# Autodesk Inventor assembly: OUTK_000_Assembly
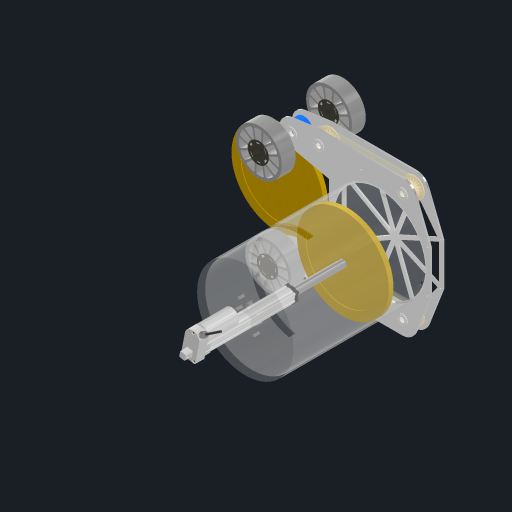
[picture p0: Inventor's stored thumbnail of the model, 512x512]
Saved by Autodesk Inventor 2024.2 (Build 282272000, 272)
## iProperties
Created: 2024-11-24
Part Number: OUTK_000_Assembly
Document SubType Name: Assembly
Designer: Bryan
Mass: 4347.94 g
Surface Area: 10314.1 cm^2
Volume: 2070.59 cm^3
Density: 2.09986 g/cm^3
Author: Bryan
## Documents named in this file (13)
- C:\Users\bobsb\OneDrive\Documents\GitHub\1622-2024-Casino-Clash-CAD-A-Thon\Outtake\OUTK_000_Assembly.iam
- C:\Users\bobsb\OneDrive\Documents\GitHub\1622-2024-Casino-Clash-CAD-A-Thon\Outtake\OUTK_002_ShotPlateNoReceptacle.ipt
- C:\Users\bobsb\OneDrive\Documents\GitHub\1622-2024-Casino-Clash-CAD-A-Thon\Outtake\OUTK_002_ShotPlateReceptacle.ipt
- C:\Users\bobsb\OneDrive\Documents\GitHub\1622-2024-Casino-Clash-CAD-A-Thon\Outtake\OUTK_001_ChipBucket.ipt
- C:\Users\bobsb\OneDrive\Documents\GitHub\1622-2024-Casino-Clash-CAD-A-Thon\COTS Library\Motion\Linear Actuators\PA-01\COTS_PA-01.iam
- C:\Users\bobsb\OneDrive\Documents\GitHub\1622-2024-Casino-Clash-CAD-A-Thon\COTS Library\Motion\Linear Actuators\PA-01\Shaft.ipt
- C:\Users\bobsb\OneDrive\Documents\GitHub\1622-2024-Casino-Clash-CAD-A-Thon\COTS Library\Motion\Bearings\COTS_WCP-0783_1.125ODHexBearing.ipt
- C:\Users\bobsb\OneDrive\Documents\GitHub\1622-2024-Casino-Clash-CAD-A-Thon\COTS Library\Motion\Wheels\Compliant Wheels\5in compliant wheels\COTS_5 Straight Flex Wheel (.ipt
- C:\Users\bobsb\OneDrive\Documents\GitHub\1622-2024-Casino-Clash-CAD-A-Thon\COTS Library\Adapters\COTS_1_2” Hex Bore Aluminum VersaHub (217-2592)(1).ipt
- C:\Users\bobsb\OneDrive\Documents\GitHub\1622-2024-Casino-Clash-CAD-A-Thon\COTS Library\Motion\Wheels\Compliant Wheels\2in compliant wheels\0.500in hex bore\COTS_am-3462_2indiameter_0.500inhexbore_durometer50A_CompliantWheel.ipt
- C:\Users\bobsb\OneDrive\Documents\GitHub\1622-2024-Casino-Clash-CAD-A-Thon\Game Objects\Chip, Simplified.ipt
- C:\Users\bobsb\OneDrive\Documents\GitHub\1622-2024-Casino-Clash-CAD-A-Thon\Outtake\OUTK_010_Grippy.ipt
- C:\Users\bobsb\OneDrive\Documents\GitHub\1622-2024-Casino-Clash-CAD-A-Thon\Outtake\OUTK_011_Tubing.ipt
## Components (41 placed, 12 different names)
1. OUTK_002_ShotPlateNoReceptacle:1 — Mate:4, Mate:5, Mate:41, Mate:47, Mate:50, Mate:52, Mate:55, Mate:56, Mate:57, Mate:65, Mate:66, Mate:67, Mate:68, Mate:69, Mate:70, Angle:1
2. OUTK_002_ShotPlateReceptacle:1 — Mate:3, Mate:4, Mate:5, Mate:41, Mate:42, Mate:48, Mate:49, Mate:51, Mate:53, Mate:54, Mate:58, Mate:59, Mate:60, Mate:61, Mate:62, Mate:63, Mate:64, Mate:116
3. OUTK_001_ChipBucket:1 — Mate:3, Mate:42, Mate:43, Mate:44, Mate:114, Flush:1
4. COTS_PA-01:1 [sub-assembly] — Mate:43, Mate:44, Mate:46, Flush:1
5. Shaft:1 — Mate:46, Mate:115
6. COTS_WCP-0783_1.125ODHexBearing:1 — Mate:47, Mate:65, Mate:72, Mate:107
7. COTS_WCP-0783_1.125ODHexBearing:2 — Mate:48, Mate:62, Mate:74, Mate:106, Mate:108
8. COTS_WCP-0783_1.125ODHexBearing:3 — Mate:49, Mate:64, Mate:120
9. COTS_WCP-0783_1.125ODHexBearing:4 — Mate:50, Mate:66, Mate:124
10. COTS_WCP-0783_1.125ODHexBearing:5 — Mate:51, Mate:63, Mate:117
11. COTS_WCP-0783_1.125ODHexBearing:6 — Mate:52, Mate:67, Mate:123
12. COTS_WCP-0783_1.125ODHexBearing:7 — Mate:55, Mate:69, Mate:122
13. COTS_WCP-0783_1.125ODHexBearing:8 — Mate:56, Mate:68, Mate:71, Mate:110, Mate:111
14. COTS_WCP-0783_1.125ODHexBearing:9 — Mate:53, Mate:61, Mate:119
15. COTS_WCP-0783_1.125ODHexBearing:10 — Mate:54, Mate:60, Mate:73, Mate:112
16. COTS_WCP-0783_1.125ODHexBearing:11 — Mate:57, Mate:70, Mate:121
17. COTS_WCP-0783_1.125ODHexBearing:12 — Mate:58, Mate:59, Mate:118
18. COTS_5 Straight Flex Wheel (:1 — Mate:71, Mate:75, Mate:80, Mate:85, Mate:88, Mate:89, Mate:90
19. COTS_5 Straight Flex Wheel (:2 — Mate:72, Mate:76, Mate:81, Mate:86, Mate:87, Mate:94, Mate:95, Mate:96
20. COTS_5 Straight Flex Wheel (:3 — Mate:73, Mate:78, Mate:79, Mate:84, Mate:91, Mate:92, Mate:93
21. COTS_5 Straight Flex Wheel (:4 — Mate:74, Mate:77, Mate:82, Mate:83, Mate:97, Mate:98, Mate:99
22. COTS_1_2” Hex Bore Aluminum VersaHub (217-2592)(1):1 — Mate:77, Mate:82, Mate:83
23. COTS_1_2” Hex Bore Aluminum VersaHub (217-2592)(1):2 — Mate:76, Mate:81, Mate:86, Mate:87
24. COTS_1_2” Hex Bore Aluminum VersaHub (217-2592)(1):3 — Mate:78, Mate:79, Mate:84
25. COTS_1_2” Hex Bore Aluminum VersaHub (217-2592)(1):4 — Mate:75, Mate:80, Mate:85
26. COTS_1_2” Hex Bore Aluminum VersaHub (217-2592)(1):5 — Mate:88, Mate:89, Mate:90
27. COTS_1_2” Hex Bore Aluminum VersaHub (217-2592)(1):6 — Mate:91, Mate:92, Mate:93
28. COTS_1_2” Hex Bore Aluminum VersaHub (217-2592)(1):7 — Mate:94, Mate:95, Mate:96
29. COTS_1_2” Hex Bore Aluminum VersaHub (217-2592)(1):8 — Mate:97, Mate:98, Mate:99
30. COTS_am-3462_2indiameter_0.500inhexbore_durometer50A_CompliantWheel:1 — Mate:106, Mate:107, Mate:109
31. COTS_am-3462_2indiameter_0.500inhexbore_durometer50A_CompliantWheel:2 — Mate:108, Mate:109
32. COTS_am-3462_2indiameter_0.500inhexbore_durometer50A_CompliantWheel:3 — Mate:110, Mate:111, Mate:113
33. COTS_am-3462_2indiameter_0.500inhexbore_durometer50A_CompliantWheel:4 — Mate:112, Mate:113
34. Chip, Simplified:1 — Mate:114, Mate:115, Tangent:1
35. Chip, Simplified:2 — Tangent:3, Mate:116
36. OUTK_010_Grippy:1 — Mate:120, Mate:124, Mate:128
37. OUTK_010_Grippy:2 — Mate:119, Mate:122, Mate:126
38. OUTK_010_Grippy:3 — Mate:118, Mate:121, Mate:125, Tangent:4
39. OUTK_010_Grippy:4 — Mate:117, Mate:123, Mate:127, Tangent:5
40. OUTK_011_Tubing:1 — Mate:125, Mate:126, Tangent:4
41. OUTK_011_Tubing:2 — Mate:127, Mate:128, Tangent:5
## Relationships (90: Mate 84, Tangent 4, Angle 1, Flush 1)
- Mate:3: OUTK_002_ShotPlateReceptacle:1 ↔ OUTK_001_ChipBucket:1
- Mate:4: OUTK_002_ShotPlateNoReceptacle:1 ↔ OUTK_002_ShotPlateReceptacle:1
- Mate:5: OUTK_002_ShotPlateNoReceptacle:1 ↔ OUTK_002_ShotPlateReceptacle:1
- Mate:41 (30.1625 mm): OUTK_002_ShotPlateNoReceptacle:1 ↔ OUTK_002_ShotPlateReceptacle:1
- Mate:42: OUTK_002_ShotPlateReceptacle:1 ↔ OUTK_001_ChipBucket:1
- Mate:43: OUTK_001_ChipBucket:1 ↔ COTS_PA-01:1
- Mate:44: OUTK_001_ChipBucket:1 ↔ COTS_PA-01:1
- Mate:46: COTS_PA-01:1 ↔ Shaft:1
- Mate:47: OUTK_002_ShotPlateNoReceptacle:1 ↔ COTS_WCP-0783_1.125ODHexBearing:1
- Mate:48: OUTK_002_ShotPlateReceptacle:1 ↔ COTS_WCP-0783_1.125ODHexBearing:2
- Mate:49: OUTK_002_ShotPlateReceptacle:1 ↔ COTS_WCP-0783_1.125ODHexBearing:3
- Mate:50: OUTK_002_ShotPlateNoReceptacle:1 ↔ COTS_WCP-0783_1.125ODHexBearing:4
- Mate:51: OUTK_002_ShotPlateReceptacle:1 ↔ COTS_WCP-0783_1.125ODHexBearing:5
- Mate:52: OUTK_002_ShotPlateNoReceptacle:1 ↔ COTS_WCP-0783_1.125ODHexBearing:6
- Mate:53: OUTK_002_ShotPlateReceptacle:1 ↔ COTS_WCP-0783_1.125ODHexBearing:9
- Mate:54: OUTK_002_ShotPlateReceptacle:1 ↔ COTS_WCP-0783_1.125ODHexBearing:10
- Mate:55: OUTK_002_ShotPlateNoReceptacle:1 ↔ COTS_WCP-0783_1.125ODHexBearing:7
- Mate:56: OUTK_002_ShotPlateNoReceptacle:1 ↔ COTS_WCP-0783_1.125ODHexBearing:8
- Mate:57: OUTK_002_ShotPlateNoReceptacle:1 ↔ COTS_WCP-0783_1.125ODHexBearing:11
- Mate:58: OUTK_002_ShotPlateReceptacle:1 ↔ COTS_WCP-0783_1.125ODHexBearing:12
- Mate:59: OUTK_002_ShotPlateReceptacle:1 ↔ COTS_WCP-0783_1.125ODHexBearing:12
- Mate:60: OUTK_002_ShotPlateReceptacle:1 ↔ COTS_WCP-0783_1.125ODHexBearing:10
- Mate:61: OUTK_002_ShotPlateReceptacle:1 ↔ COTS_WCP-0783_1.125ODHexBearing:9
- Mate:62: OUTK_002_ShotPlateReceptacle:1 ↔ COTS_WCP-0783_1.125ODHexBearing:2
- Mate:63: OUTK_002_ShotPlateReceptacle:1 ↔ COTS_WCP-0783_1.125ODHexBearing:5
- Mate:64: OUTK_002_ShotPlateReceptacle:1 ↔ COTS_WCP-0783_1.125ODHexBearing:3
- Mate:65: OUTK_002_ShotPlateNoReceptacle:1 ↔ COTS_WCP-0783_1.125ODHexBearing:1
- Mate:66: OUTK_002_ShotPlateNoReceptacle:1 ↔ COTS_WCP-0783_1.125ODHexBearing:4
- Mate:67: OUTK_002_ShotPlateNoReceptacle:1 ↔ COTS_WCP-0783_1.125ODHexBearing:6
- Mate:68: OUTK_002_ShotPlateNoReceptacle:1 ↔ COTS_WCP-0783_1.125ODHexBearing:8
- Mate:69: OUTK_002_ShotPlateNoReceptacle:1 ↔ COTS_WCP-0783_1.125ODHexBearing:7
- Mate:70: OUTK_002_ShotPlateNoReceptacle:1 ↔ COTS_WCP-0783_1.125ODHexBearing:11
- Mate:71: COTS_WCP-0783_1.125ODHexBearing:8 ↔ COTS_5 Straight Flex Wheel (:1
- Mate:72: COTS_WCP-0783_1.125ODHexBearing:1 ↔ COTS_5 Straight Flex Wheel (:2
- Mate:73: COTS_WCP-0783_1.125ODHexBearing:10 ↔ COTS_5 Straight Flex Wheel (:3
- Mate:74: COTS_WCP-0783_1.125ODHexBearing:2 ↔ COTS_5 Straight Flex Wheel (:4
- Mate:75: COTS_5 Straight Flex Wheel (:1 ↔ COTS_1_2” Hex Bore Aluminum VersaHub (217-2592)(1):4
- Mate:76: COTS_5 Straight Flex Wheel (:2 ↔ COTS_1_2” Hex Bore Aluminum VersaHub (217-2592)(1):2
- Mate:77: COTS_5 Straight Flex Wheel (:4 ↔ COTS_1_2” Hex Bore Aluminum VersaHub (217-2592)(1):1
- Mate:78: COTS_5 Straight Flex Wheel (:3 ↔ COTS_1_2” Hex Bore Aluminum VersaHub (217-2592)(1):3
- Mate:79: COTS_5 Straight Flex Wheel (:3 ↔ COTS_1_2” Hex Bore Aluminum VersaHub (217-2592)(1):3
- Mate:80: COTS_5 Straight Flex Wheel (:1 ↔ COTS_1_2” Hex Bore Aluminum VersaHub (217-2592)(1):4
- Mate:81: COTS_5 Straight Flex Wheel (:2 ↔ COTS_1_2” Hex Bore Aluminum VersaHub (217-2592)(1):2
- Mate:82: COTS_5 Straight Flex Wheel (:4 ↔ COTS_1_2” Hex Bore Aluminum VersaHub (217-2592)(1):1
- Mate:83: COTS_5 Straight Flex Wheel (:4 ↔ COTS_1_2” Hex Bore Aluminum VersaHub (217-2592)(1):1
- Mate:84: COTS_5 Straight Flex Wheel (:3 ↔ COTS_1_2” Hex Bore Aluminum VersaHub (217-2592)(1):3
- Mate:85: COTS_5 Straight Flex Wheel (:1 ↔ COTS_1_2” Hex Bore Aluminum VersaHub (217-2592)(1):4
- Mate:86: COTS_5 Straight Flex Wheel (:2 ↔ COTS_1_2” Hex Bore Aluminum VersaHub (217-2592)(1):2
- Mate:87: COTS_5 Straight Flex Wheel (:2 ↔ COTS_1_2” Hex Bore Aluminum VersaHub (217-2592)(1):2
- Mate:88: COTS_5 Straight Flex Wheel (:1 ↔ COTS_1_2” Hex Bore Aluminum VersaHub (217-2592)(1):5
- Mate:89: COTS_5 Straight Flex Wheel (:1 ↔ COTS_1_2” Hex Bore Aluminum VersaHub (217-2592)(1):5
- Mate:90: COTS_5 Straight Flex Wheel (:1 ↔ COTS_1_2” Hex Bore Aluminum VersaHub (217-2592)(1):5
- Mate:91: COTS_5 Straight Flex Wheel (:3 ↔ COTS_1_2” Hex Bore Aluminum VersaHub (217-2592)(1):6
- Mate:92: COTS_5 Straight Flex Wheel (:3 ↔ COTS_1_2” Hex Bore Aluminum VersaHub (217-2592)(1):6
- Mate:93: COTS_5 Straight Flex Wheel (:3 ↔ COTS_1_2” Hex Bore Aluminum VersaHub (217-2592)(1):6
- Mate:94: COTS_5 Straight Flex Wheel (:2 ↔ COTS_1_2” Hex Bore Aluminum VersaHub (217-2592)(1):7
- Mate:95: COTS_5 Straight Flex Wheel (:2 ↔ COTS_1_2” Hex Bore Aluminum VersaHub (217-2592)(1):7
- Mate:96: COTS_5 Straight Flex Wheel (:2 ↔ COTS_1_2” Hex Bore Aluminum VersaHub (217-2592)(1):7
- Mate:97: COTS_5 Straight Flex Wheel (:4 ↔ COTS_1_2” Hex Bore Aluminum VersaHub (217-2592)(1):8
- Mate:98: COTS_5 Straight Flex Wheel (:4 ↔ COTS_1_2” Hex Bore Aluminum VersaHub (217-2592)(1):8
- Mate:99: COTS_5 Straight Flex Wheel (:4 ↔ COTS_1_2” Hex Bore Aluminum VersaHub (217-2592)(1):8
- Mate:106: COTS_WCP-0783_1.125ODHexBearing:2 ↔ COTS_am-3462_2indiameter_0.500inhexbore_durometer50A_CompliantWheel:1
- Mate:107 (0.7937 mm): COTS_WCP-0783_1.125ODHexBearing:1 ↔ COTS_am-3462_2indiameter_0.500inhexbore_durometer50A_CompliantWheel:1
- Mate:108: COTS_WCP-0783_1.125ODHexBearing:2 ↔ COTS_am-3462_2indiameter_0.500inhexbore_durometer50A_CompliantWheel:2
- Mate:109: COTS_am-3462_2indiameter_0.500inhexbore_durometer50A_CompliantWheel:1 ↔ COTS_am-3462_2indiameter_0.500inhexbore_durometer50A_CompliantWheel:2
- Mate:110: COTS_WCP-0783_1.125ODHexBearing:8 ↔ COTS_am-3462_2indiameter_0.500inhexbore_durometer50A_CompliantWheel:3
- Mate:111 (0.7937 mm): COTS_WCP-0783_1.125ODHexBearing:8 ↔ COTS_am-3462_2indiameter_0.500inhexbore_durometer50A_CompliantWheel:3
- Mate:112: COTS_WCP-0783_1.125ODHexBearing:10 ↔ COTS_am-3462_2indiameter_0.500inhexbore_durometer50A_CompliantWheel:4
- Mate:113: COTS_am-3462_2indiameter_0.500inhexbore_durometer50A_CompliantWheel:3 ↔ COTS_am-3462_2indiameter_0.500inhexbore_durometer50A_CompliantWheel:4
- Mate:114: OUTK_001_ChipBucket:1 ↔ Chip, Simplified:1
- Mate:115: Shaft:1 ↔ Chip, Simplified:1
- Angle:1 (0 deg): OUTK_002_ShotPlateNoReceptacle:1
- Tangent:1: Chip, Simplified:1
- Tangent:3: Chip, Simplified:2
- Mate:116 (8.7313 mm): OUTK_002_ShotPlateReceptacle:1 ↔ Chip, Simplified:2
- Flush:1 (15.875 mm): OUTK_001_ChipBucket:1 ↔ COTS_PA-01:1
- Mate:117: COTS_WCP-0783_1.125ODHexBearing:5 ↔ OUTK_010_Grippy:4
- Mate:118: COTS_WCP-0783_1.125ODHexBearing:12 ↔ OUTK_010_Grippy:3
- Mate:119: COTS_WCP-0783_1.125ODHexBearing:9 ↔ OUTK_010_Grippy:2
- Mate:120: COTS_WCP-0783_1.125ODHexBearing:3 ↔ OUTK_010_Grippy:1
- Mate:121 (0.7937 mm): COTS_WCP-0783_1.125ODHexBearing:11 ↔ OUTK_010_Grippy:3
- Mate:122 (0.7937 mm): COTS_WCP-0783_1.125ODHexBearing:7 ↔ OUTK_010_Grippy:2
- Mate:123 (0.7937 mm): COTS_WCP-0783_1.125ODHexBearing:6 ↔ OUTK_010_Grippy:4
- Mate:124 (0.7937 mm): COTS_WCP-0783_1.125ODHexBearing:4 ↔ OUTK_010_Grippy:1
- Mate:125: OUTK_010_Grippy:3 ↔ OUTK_011_Tubing:1
- Mate:126: OUTK_010_Grippy:2 ↔ OUTK_011_Tubing:1
- Tangent:4: OUTK_010_Grippy:3 ↔ OUTK_011_Tubing:1
- Mate:127: OUTK_010_Grippy:4 ↔ OUTK_011_Tubing:2
- Mate:128: OUTK_010_Grippy:1 ↔ OUTK_011_Tubing:2
- Tangent:5: OUTK_010_Grippy:4 ↔ OUTK_011_Tubing:2
